# Autodesk Inventor assembly: FE-00017
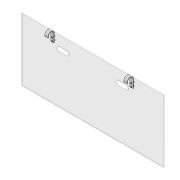
[picture p0: Inventor's stored thumbnail of the model, 180x180]
Saved by Autodesk Inventor 2012 (Build 160160000, 160)
## iProperties
Created: 2008-06-03
Part Number: FE-00017
Document SubType Name: Assembly
Designer: mcyr
Author: mcyr
## Documents named in this file (5)
- C:\Data Folder\FRC 2012 Field\Components\FE-00017.iam
- C:\Data Folder\FRC 2012 Field\Components\FE-00011.ipt
- C:\Data Folder\FRC 2012 Field\Components\FE-00016.ipt
- C:\Data Folder\FRC 2012 Field\Components\HW-00002.ipt
- C:\Data Folder\FRC 2012 Field\Components\HW-00012.ipt
## Components (11 placed, 4 different names)
1. FE-00011:1 — Mate:1, Mate:2, Mate:3, Mate:4, Mate:9, Mate:11, Mate:14, Mate:17, Mate:19
2. FE-00016:1 — Mate:1, Mate:2, Mate:5, Mate:6, Mate:7, Mate:8
3. FE-00016:2 — Mate:3, Mate:4, Mate:13, Mate:15, Mate:16
4. HW-00002:1 — Mate:9, Mate:10
5. HW-00002:2 — Mate:11, Mate:12
6. HW-00002:3 — Mate:19, Mate:20
7. HW-00002:4 — Mate:17, Mate:18
8. HW-00012:1 — Mate:5, Mate:7, Mate:10
9. HW-00012:2 — Mate:6, Mate:8, Mate:12
10. HW-00012:3 — Mate:13, Mate:16, Mate:20
11. HW-00012:4 — Mate:14, Mate:15, Mate:18
## Relationships (20: Mate 20)
- Mate:1: FE-00011:1 ↔ FE-00016:1
- Mate:2: FE-00011:1 ↔ FE-00016:1
- Mate:3: FE-00011:1 ↔ FE-00016:2
- Mate:4: FE-00011:1 ↔ FE-00016:2
- Mate:5: FE-00016:1 ↔ HW-00012:1
- Mate:6: FE-00016:1 ↔ HW-00012:2
- Mate:7: FE-00016:1 ↔ HW-00012:1
- Mate:8: FE-00016:1 ↔ HW-00012:2
- Mate:9: FE-00011:1 ↔ HW-00002:1
- Mate:10: HW-00002:1 ↔ HW-00012:1
- Mate:11: FE-00011:1 ↔ HW-00002:2
- Mate:12: HW-00002:2 ↔ HW-00012:2
- Mate:13: FE-00016:2 ↔ HW-00012:3
- Mate:14: FE-00011:1 ↔ HW-00012:4
- Mate:15: FE-00016:2 ↔ HW-00012:4
- Mate:16: FE-00016:2 ↔ HW-00012:3
- Mate:17: FE-00011:1 ↔ HW-00002:4
- Mate:18: HW-00002:4 ↔ HW-00012:4
- Mate:19: FE-00011:1 ↔ HW-00002:3
- Mate:20: HW-00002:3 ↔ HW-00012:3
